# Autodesk Inventor assembly: tractor
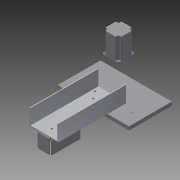
[picture p0: Inventor's stored thumbnail of the model, 180x180]
Saved by Autodesk Inventor 2013 (Build 170138000, 138)
## iProperties
Created: 2012-11-28
Part Number: tractor
Document SubType Name: Assembly
Designer: istvan.burbank
Mass: 847.083 g
Surface Area: 1890.52 cm^2
Volume: 847.083 cm^3
Density: 1 g/cm^3
Author: istvan.burbank
## Documents named in this file (7)
- C:\Users\istvan.burbank\Documents\GitHub\Crown-Fire\CAD\GantryMount\tractor.iam
- C:\Users\istvan.burbank\Documents\GitHub\Crown-Fire\CAD\GantryMount\tractor.ipt
- C:\Users\istvan.burbank\Documents\GitHub\Crown-Fire\CAD\Electronics\Motors\G723-280-4.ipt
- C:\Users\istvan.burbank\Documents\GitHub\Crown-Fire\CAD\Hardware\Bearings\DualVee-size2.ipt
- C:\Users\istvan.burbank\Documents\GitHub\Crown-Fire\CAD\GantryMount\gantryMount.ipt
- C:\Users\istvan.burbank\Documents\GitHub\Crown-Fire\CAD\GantryMount\channelRack.ipt
- C:\Users\istvan.burbank\Documents\GitHub\Crown-Fire\CAD\Templates\channel2.25x4.ipt
## Components (6 placed, 5 different names)
1. tractor:1 — Mate:4, Mate:5, Mate:6, Flush:3
2. G723-280-4:1
3. DualVee-size2:1 — Mate:5, Flush:1
4. DualVee-size2:2 — Mate:4, Flush:1
5. gantryMount:1 — Flush:2
6. channelRack:2 — Mate:6, Flush:2, Flush:3
## Relationships (6: Mate 3, Flush 3)
- Mate:4: tractor:1 ↔ DualVee-size2:2
- Mate:5: tractor:1 ↔ DualVee-size2:1
- Flush:1: DualVee-size2:1 ↔ DualVee-size2:2
- Mate:6: tractor:1 ↔ channelRack:2
- Flush:2: gantryMount:1 ↔ channelRack:2
- Flush:3 (76.2 mm): tractor:1 ↔ channelRack:2
